# Autodesk Inventor assembly: robot v11 final frame for may
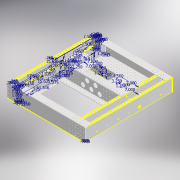
[picture p0: Inventor's stored thumbnail of the model, 180x180]
Saved by Autodesk Inventor 2022 (Build 260153000, 153)
## iProperties
Created: 2022-01-17
Part Number: robot v11 final frame for may
Document SubType Name: Assembly
Designer: 5126_Cad_2
Author: 5126_Cad_2
## Documents named in this file (12)
- A:\robot v11 final frame for may.iam
- A:\new 2022 cad\new 2022 cad\front-back pannel 00000.ipt
- A:\new 2022 cad\new 2022 cad\side with gearbox.iam
- A:\new 2022 cad\new 2022 cad\side with gearbox_MIR1.iam
- A:\new 2022 cad\new 2022 cad\drive train parts\side pannel 1 00001_MIR.ipt
- A:\new 2022 cad\new 2022 cad\s flange 1.ipt
- A:\new 2022 cad\new 2022 cad\s flange 2.ipt
- A:\new 2022 cad\new 2022 cad\side pannel 1 00001.ipt
- side pannel 1 00001.ipt
- A:\new 2022 cad\new 2022 cad\side with gearbox_MIR5.iam
- A:\new 2022 cad\new 2022 cad\side pannel 1 00001_MIR1.ipt
- A:\new 2022 cad\new 2022 cad\top plate 3.ipt
## Components (11 placed, 10 different names)
1. front-back pannel 00000:1 — Mate:326, Mate:328, Mate:329, Mate:330, Mate:331, Mate:344, Mate:387, Mate:388, Mate:402, Mate:403
2. front-back pannel 00000:2 — Mate:131, Mate:325, Mate:334, Mate:335, Mate:336, Mate:337, Mate:338, Mate:339, Mate:383, Mate:384, Mate:385, Mate:386, Mate:401, Mate:404
3. side with gearbox:1 [sub-assembly] — Mate:325, Mate:329, Mate:330, Mate:331, Mate:336, Mate:337, Mate:338, Mate:341, Mate:342, Mate:343, Mate:396, Mate:397, Mate:399, Mate:400, Mate:401, Mate:402
4. side with gearbox_MIR1:1 [sub-assembly]
5. side pannel 1 00001_MIR:1 — Mate:130
6. s flange 1:1 — Mate:341, Mate:342, Mate:343
7. s flange 2:1 — Mate:398, Mate:399, Mate:400
8. side pannel 1 00001:1 — Mate:326, Mate:328, Mate:334, Mate:335, Mate:339, Mate:344, Mate:405
9. side with gearbox_MIR5:1 [sub-assembly] — Mate:385, Mate:386, Mate:387, Mate:395, Mate:403
10. side pannel 1 00001_MIR1:1 — Mate:383, Mate:384, Mate:388
11. top plate 3:1 — Mate:395, Mate:396, Mate:397, Mate:398
## Relationships (35: Mate 35)
- Mate:130 (-355.6 mm): side pannel 1 00001_MIR:1
- Mate:131: front-back pannel 00000:2
- Mate:325: front-back pannel 00000:2 ↔ side with gearbox:1
- Mate:326: front-back pannel 00000:1 ↔ side pannel 1 00001:1
- Mate:328: front-back pannel 00000:1 ↔ side pannel 1 00001:1
- Mate:329: front-back pannel 00000:1 ↔ side with gearbox:1
- Mate:330: front-back pannel 00000:1 ↔ side with gearbox:1
- Mate:331: front-back pannel 00000:1 ↔ side with gearbox:1
- Mate:334: front-back pannel 00000:2 ↔ side pannel 1 00001:1
- Mate:335: front-back pannel 00000:2 ↔ side pannel 1 00001:1
- Mate:336: front-back pannel 00000:2 ↔ side with gearbox:1
- Mate:337: front-back pannel 00000:2 ↔ side with gearbox:1
- Mate:338: front-back pannel 00000:2 ↔ side with gearbox:1
- Mate:339: front-back pannel 00000:2 ↔ side pannel 1 00001:1
- Mate:341: side with gearbox:1 ↔ s flange 1:1
- Mate:342: side with gearbox:1 ↔ s flange 1:1
- Mate:343: side with gearbox:1 ↔ s flange 1:1
- Mate:344: front-back pannel 00000:1 ↔ side pannel 1 00001:1
- Mate:383: front-back pannel 00000:2 ↔ side pannel 1 00001_MIR1:1
- Mate:384: front-back pannel 00000:2 ↔ side pannel 1 00001_MIR1:1
- Mate:385: front-back pannel 00000:2 ↔ side with gearbox_MIR5:1
- Mate:386: front-back pannel 00000:2 ↔ side with gearbox_MIR5:1
- Mate:387: front-back pannel 00000:1 ↔ side with gearbox_MIR5:1
- Mate:388: front-back pannel 00000:1 ↔ side pannel 1 00001_MIR1:1
- Mate:395: side with gearbox_MIR5:1 ↔ top plate 3:1
- Mate:396: side with gearbox:1 ↔ top plate 3:1
- Mate:397: side with gearbox:1 ↔ top plate 3:1
- Mate:398: s flange 2:1 ↔ top plate 3:1
- Mate:399: side with gearbox:1 ↔ s flange 2:1
- Mate:400: side with gearbox:1 ↔ s flange 2:1
- Mate:401: front-back pannel 00000:2 ↔ side with gearbox:1
- Mate:402: front-back pannel 00000:1 ↔ side with gearbox:1
- Mate:403: front-back pannel 00000:1 ↔ side with gearbox_MIR5:1
- Mate:404: front-back pannel 00000:2
- Mate:405: side pannel 1 00001:1
